# Autodesk Inventor assembly: ZSB_210324
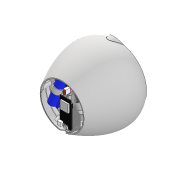
[picture p0: Inventor's stored thumbnail of the model, 180x180]
Saved by Autodesk Inventor 2020 (Build 240168000, 168)
## iProperties
Created: 2021-03-24
Part Number: ZSB_210324
Document SubType Name: Assembly
Designer: uhlma
Author: uhlma
## Documents named in this file (11)
- C:\Users\uhlma\OneDrive\Flaura\Produktentwicklung\Gehaeuse\CAD-Konstruktion\Prototyp 9\Thingiverse_Upload\Inventor\Assambly_Flaura.iam
- C:\Users\uhlma\OneDrive\Flaura\Produktentwicklung\Gehaeuse\CAD-Konstruktion\Prototyp 9\Thingiverse_Upload\Inventor\Dummy_ESP32_WEMOS_LOLIN32.ipt
- C:\Users\uhlma\OneDrive\Flaura\Produktentwicklung\Gehaeuse\CAD-Konstruktion\Prototyp 9\Thingiverse_Upload\Inventor\Dummy_Water_Pump.ipt
- C:\Users\uhlma\OneDrive\Flaura\Produktentwicklung\Gehaeuse\CAD-Konstruktion\Prototyp 9\Thingiverse_Upload\Inventor\Dummy_Capacitive_Soil_Sensor.ipt
- C:\Users\uhlma\OneDrive\Flaura\Produktentwicklung\Gehaeuse\CAD-Konstruktion\Prototyp 9\Thingiverse_Upload\Inventor\Dummy_LiPo_Battery_18650.ipt
- C:\Users\uhlma\OneDrive\Flaura\Produktentwicklung\Gehaeuse\CAD-Konstruktion\Prototyp 9\Thingiverse_Upload\Inventor\Dummy_Circuit_Board.ipt
- C:\Users\uhlma\OneDrive\Flaura\Produktentwicklung\Gehaeuse\CAD-Konstruktion\Prototyp 9\Thingiverse_Upload\Inventor\Water_Level_Sensor_Mount.ipt
- C:\Users\uhlma\OneDrive\Flaura\Produktentwicklung\Gehaeuse\CAD-Konstruktion\Prototyp 9\Thingiverse_Upload\Inventor\Battery_Mount.ipt
- C:\Users\uhlma\OneDrive\Flaura\Produktentwicklung\Gehaeuse\CAD-Konstruktion\Prototyp 9\Thingiverse_Upload\Inventor\Water_Pump_Mount.ipt
- C:\Users\uhlma\OneDrive\Flaura\Produktentwicklung\Gehaeuse\CAD-Konstruktion\Prototyp 9\Thingiverse_Upload\Inventor\Housing_Bottom.ipt
- C:\Users\uhlma\OneDrive\Flaura\Produktentwicklung\Gehaeuse\CAD-Konstruktion\Prototyp 9\Thingiverse_Upload\Inventor\Housing_Inner_Outer.ipt
## Components (10 placed, 10 different names)
1. Housing_Inner_Outer:1 — Passend:1
2. Housing_Bottom:1 — Passend:1, Passend:2, Passend:3, Passend:36, Passend:37, Winkel:5, Einfügen:10, Passend:45, Einfügen:11, Einfügen:12, Einfügen:13, Einfügen:14, Passend:46
3. Dummy_Water_Pump:1 — Passend:41
4. Dummy_Capacitive_Soil_Sensor:1 — Fluchtend:40, Passend:45, Passend:46
5. Dummy_ESP32_WEMOS_LOLIN32:2 — Fluchtend:33, Passend:30, Fluchtend:34
6. Dummy_LiPo_Battery_18650:1 — Passend:40
7. Dummy_Circuit_Board:1 — Fluchtend:30, Fluchtend:31, Passend:29, Fluchtend:33, Passend:30, Fluchtend:34, Fluchtend:35, Fluchtend:41
8. Water_Pump_Mount:1 — Passend:41, Einfügen:13, Einfügen:14
9. Battery_Mount:1 — Passend:40, Einfügen:11, Einfügen:12
10. Water_Level_Sensor_Mount:1 — Einfügen:10
## Relationships (25: Mate 11, Flush 8, Insert 5, Angle 1)
- Passend:1 [Mate]: Housing_Inner_Outer:1 ↔ Housing_Bottom:1
- Passend:2 [Mate]: Housing_Bottom:1
- Passend:3 [Mate]: Housing_Bottom:1
- Fluchtend:30 [Flush] (-15.1 mm): Dummy_Circuit_Board:1
- Fluchtend:31 [Flush] (19.35 mm): Dummy_Circuit_Board:1
- Fluchtend:32 [Flush]
- Passend:29 [Mate] (-3.6 mm): Dummy_Circuit_Board:1
- Fluchtend:33 [Flush]: Dummy_ESP32_WEMOS_LOLIN32:2 ↔ Dummy_Circuit_Board:1
- Passend:30 [Mate]: Dummy_ESP32_WEMOS_LOLIN32:2 ↔ Dummy_Circuit_Board:1
- Fluchtend:34 [Flush]: Dummy_ESP32_WEMOS_LOLIN32:2 ↔ Dummy_Circuit_Board:1
- Fluchtend:35 [Flush]: Dummy_Circuit_Board:1
- Passend:36 [Mate]: Housing_Bottom:1
- Passend:37 [Mate]: Housing_Bottom:1
- Winkel:5 [Angle] (0 deg): Housing_Bottom:1
- Fluchtend:40 [Flush]: Dummy_Capacitive_Soil_Sensor:1
- Fluchtend:41 [Flush] (1.6 mm): Dummy_Circuit_Board:1
- Einfügen:10 [Insert]: Housing_Bottom:1 ↔ Water_Level_Sensor_Mount:1
- Passend:40 [Mate]: Dummy_LiPo_Battery_18650:1 ↔ Battery_Mount:1
- Passend:41 [Mate]: Dummy_Water_Pump:1 ↔ Water_Pump_Mount:1
- Passend:45 [Mate]: Housing_Bottom:1 ↔ Dummy_Capacitive_Soil_Sensor:1
- Einfügen:11 [Insert]: Housing_Bottom:1 ↔ Battery_Mount:1
- Einfügen:12 [Insert]: Housing_Bottom:1 ↔ Battery_Mount:1
- Einfügen:13 [Insert]: Housing_Bottom:1 ↔ Water_Pump_Mount:1
- Einfügen:14 [Insert]: Housing_Bottom:1 ↔ Water_Pump_Mount:1
- Passend:46 [Mate] (0.25 mm): Housing_Bottom:1 ↔ Dummy_Capacitive_Soil_Sensor:1
